# Autodesk Inventor assembly: ASY NDM 11.025 перегородка рама 1.1  вертикал
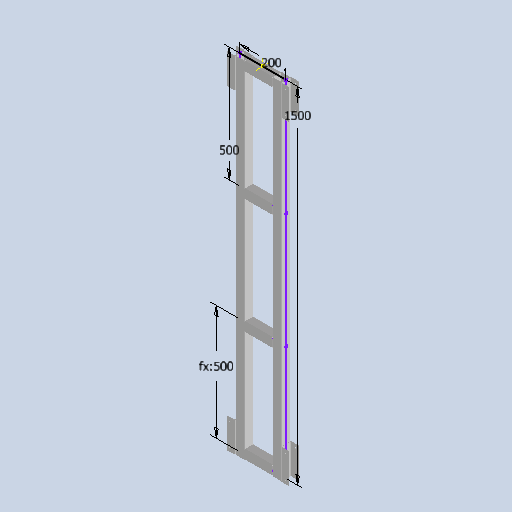
[picture p0: Inventor's stored thumbnail of the model, 512x512]
Saved by Autodesk Inventor 2025 (Build 290162010, 162A)
## iProperties
_SolveAssemblyDoc: Frame Generator Solve Assembly
_Version: 25.0.0
Created: 2024-08-18
Part Number: ASY NDM 11.025 перегородка рама 1.1  вертикал
Document SubType Name: Assembly
Designer: admin
Author: admin
## Documents named in this file (4)
- C:\Users\admin\YandexDisk-badmisterfox\домашниий пк\Inventor\Nadyim\CAD\Перегородка\ASY NDM 11.025 перегородка рама 1.1  вертикал.iam
- C:\Users\admin\YandexDisk-badmisterfox\домашниий пк\Inventor\Nadyim\ASY NDM 11.024 перегородка рама 1.1  вертикал.ipt
- C:\Users\admin\YandexDisk-badmisterfox\домашниий пк\Inventor\Nadyim\CAD\Перегородка\ASY NDM 11.025 перегородка рама 1.1  вертикал\Frame\Frame 1723967280938.iam
- C:\Users\admin\YandexDisk-badmisterfox\домашниий пк\Inventor\Nadyim\CAD\кронштейн\NDM 11.027 кронштейн 27.ipt
## Components (6 placed, 3 different names)
1. ASY NDM 11.024 перегородка рама 1.1  вертикал:1
2. Frame 1723967280938:1 [sub-assembly] — Rigid:1, Rigid:2, Rigid:3, Rigid:4
3. NDM 11.027 кронштейн 27:1 — Rigid:1
4. NDM 11.027 кронштейн 27:2 — Rigid:2
5. NDM 11.027 кронштейн 27:3 — Rigid:3
6. NDM 11.027 кронштейн 27:4 — Rigid:4
## Relationships (4: WeldJoint 4)
- Rigid:1 [WeldJoint]: Frame 1723967280938:1 ↔ NDM 11.027 кронштейн 27:1
- Rigid:2 [WeldJoint]: Frame 1723967280938:1 ↔ NDM 11.027 кронштейн 27:2
- Rigid:3 [WeldJoint]: Frame 1723967280938:1 ↔ NDM 11.027 кронштейн 27:3
- Rigid:4 [WeldJoint]: Frame 1723967280938:1 ↔ NDM 11.027 кронштейн 27:4
